# Autodesk Inventor assembly: BoxBeamDBAssembly
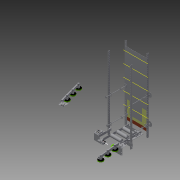
[picture p0: Inventor's stored thumbnail of the model, 180x180]
Saved by Autodesk Inventor 2015 (Build 190159000, 159)
## iProperties
Created: 2015-01-18
Part Number: BoxBeamDBAssembly
Document SubType Name: Assembly
Designer: whitaus15
Author: whitaus15
Title: \\lhssvr02\Homedirs\Robotics Club\CAD Model 2015\Box Beam Drive Base\BoxBeamDBAssembly.stp
Creation Date: 2015-01-17
Sending System: Autodesk Inventor 2015
Preprocessor: ST-DEVELOPER v15.6
## Documents named in this file (21)
- \\lhssvr02\Homedirs\Robotics Club\CAD Model 2015\Box Beam Drive Base\BoxBeamDBAssembly.iam
- \\lhssvr02\Homedirs\Robotics Club\CAD Model 2015\Box Beam Drive Base\Imported Components\BoxBeamDBAssembly\c hannel.ipt
- \\lhssvr02\Homedirs\Robotics Club\CAD Model 2015\Box Beam Drive Base\Imported Components\BoxBeamDBAssembly\Elevator Sprocket with Sprockets.iam
- \\lhssvr02\Homedirs\Robotics Club\CAD Model 2015\Box Beam Drive Base\Imported Components\BoxBeamDBAssembly\c hannel_MIR6.ipt
- \\lhssvr02\Homedirs\Robotics Club\CAD Model 2015\Box Beam Drive Base\Imported Components\BoxBeamDBAssembly\Elevator Sprocket with Sprockets_MIR3.iam
- \\lhssvr02\Homedirs\Robotics Club\CAD Model 2015\Fc Fender Assembly_MIR5.iam
- \\lhssvr02\Homedirs\Robotics Club\CAD Model 2015\Bearing plate version 2.0_MIR4.ipt
- \\lhssvr02\Homedirs\Robotics Club\CAD Model 2015\Fender and Igus.iam
- \\lhssvr02\Homedirs\Robotics Club\CAD Model 2015\Front bar with Motors.iam
- \\lhssvr02\Homedirs\Robotics Club\CAD Model 2015\Fc Fender Assembly_MIR5_MIR.iam
- \\lhssvr02\Homedirs\Robotics Club\CAD Model 2015\Bearing plate version 2.0_MIR4_MIR.ipt
- \\lhssvr02\Homedirs\Robotics Club\CAD Model 2015\Fender and Igus_MIR3.iam
- \\lhssvr02\Homedirs\Robotics Club\CAD Model 2015\Front bar with Motors_MIR.iam
- \\lhssvr02\Homedirs\Robotics Club\CAD Model 2015\Box Beam Drive Base\Conveyor.iam
- \\lhssvr02\Homedirs\Robotics Club\CAD Model 2015\Box Beam Drive Base\Imported Components\BoxBeamDBAssembly\c hannel_MIR.ipt
- \\lhssvr02\Homedirs\Robotics Club\CAD Model 2015\Box Beam Drive Base\Back plate.ipt
- \\lhssvr02\Homedirs\Robotics Club\CAD Model 2015\Box Beam Drive Base\electronics board.iam
- \\lhssvr02\Homedirs\Robotics Club\CAD Model 2015\Elevator parts\Gearbox\Elevator Gearbox Assembly.iam
- \\lhssvr02\Homedirs\Robotics Club\CAD Model 2015\Box Beam Drive Base\Newest\Elevator Shaft Mounts.ipt
- \\lhssvr02\Homedirs\Robotics Club\CAD Model 2015\Elevator parts\Gearbox\S25-60L Aluminum Sprocket (am-0237).0002.ipt
- \\lhssvr02\Homedirs\Robotics Club\CAD Model 2015\Elevator parts\Gearbox\22 tooth sprocket.ipt
## Components (35 placed, 20 different names)
1. c hannel:2 — Angle:2, Mate:12, Mate:19, Mate:22, Mate:23, Mate:53, Mate:57
2. c hannel:3 — Mate:20, Mate:21, Mate:24, Mate:41, Mate:54, Mate:55
3. Elevator Sprocket with Sprockets:1 [sub-assembly] — Mate:30, Mate:61
4. Elevator Sprocket with Sprockets:2 [sub-assembly] — Mate:45, Mate:58, Mate:59
5. c hannel_MIR6:1 — Mate:17, Mate:28, Mate:29, Mate:36, Mate:37, Mate:38
6. Elevator Sprocket with Sprockets_MIR3:1 [sub-assembly] — Mate:25, Mate:64
7. Elevator Sprocket with Sprockets_MIR3:2 [sub-assembly] — Mate:35, Mate:60
8. Fc Fender Assembly_MIR5:1 [sub-assembly] — Flush:10, Flush:11, Mate:15
9. Front bar with Motors:1 [sub-assembly] — Mate:11, Flush:8
10. Fc Fender Assembly_MIR5_MIR:1 [sub-assembly]
11. Bearing plate version 2.0_MIR4_MIR:1 — Mate:8, Mate:9
12. Fender and Igus_MIR3:1 [sub-assembly] — Mate:8, Mate:9
13. Front bar with Motors_MIR:1 [sub-assembly]
14. Back plate:1 — Angle:2, Mate:12, Mate:16, Mate:32, Mate:33, Mate:48, Mate:56
15. Conveyor:1 [sub-assembly] — Mate:11, Flush:8
16. c hannel_MIR:1 — Mate:13, Mate:18, Mate:26, Mate:27, Mate:39
17. electronics board:1 [sub-assembly] — Mate:13, Mate:34, Mate:53, Mate:62, Mate:63
18. Bearing plate version 2.0_MIR4:1
19. Fender and Igus:1 [sub-assembly]
20. Bearing plate version 2.0_MIR4:2 — Flush:10, Flush:11, Mate:15
21. Elevator Gearbox Assembly:1 [sub-assembly] — Mate:16
22. Elevator Shaft Mounts:1 — Mate:18, Mate:26, Mate:27, Mate:30
23. Elevator Shaft Mounts:2 — Mate:17, Mate:28, Mate:29
24. Elevator Shaft Mounts:3 — Mate:19, Mate:22, Mate:23, Mate:25
25. Elevator Shaft Mounts:4 — Mate:20, Mate:21, Mate:24
26. Elevator Shaft Mounts:5 — Mate:32, Mate:33, Mate:34, Mate:35, Mate:39
27. Elevator Shaft Mounts:6 — Mate:36, Mate:37, Mate:38
28. Elevator Shaft Mounts:7 — Mate:41, Mate:54, Mate:55, Mate:58
29. Elevator Shaft Mounts:8 — Mate:45, Mate:48, Mate:56, Mate:57
30. S25-60L Aluminum Sprocket (am-0237).0002:1 — Mate:59
31. S25-60L Aluminum Sprocket (am-0237).0002:2 — Mate:60
32. 22 tooth sprocket:1 — Mate:63
33. 22 tooth sprocket:2 — Mate:62
34. S25-60L Aluminum Sprocket (am-0237).0002:3 — Mate:64
35. S25-60L Aluminum Sprocket (am-0237).0002:4 — Mate:61
## Relationships (48: Mate 44, Flush 3, Angle 1)
- Mate:8: Bearing plate version 2.0_MIR4_MIR:1 ↔ Fender and Igus_MIR3:1
- Mate:9: Bearing plate version 2.0_MIR4_MIR:1 ↔ Fender and Igus_MIR3:1
- Mate:11: Front bar with Motors:1 ↔ Conveyor:1
- Flush:8: Front bar with Motors:1 ↔ Conveyor:1
- Angle:2 (0 deg): c hannel:2 ↔ Back plate:1
- Mate:12: c hannel:2 ↔ Back plate:1
- Mate:13: c hannel_MIR:1 ↔ electronics board:1
- Flush:10: Fc Fender Assembly_MIR5:1 ↔ Bearing plate version 2.0_MIR4:2
- Flush:11: Fc Fender Assembly_MIR5:1 ↔ Bearing plate version 2.0_MIR4:2
- Mate:15: Fc Fender Assembly_MIR5:1 ↔ Bearing plate version 2.0_MIR4:2
- Mate:16: Back plate:1 ↔ Elevator Gearbox Assembly:1
- Mate:17: c hannel_MIR6:1 ↔ Elevator Shaft Mounts:2
- Mate:18: c hannel_MIR:1 ↔ Elevator Shaft Mounts:1
- Mate:19: c hannel:2 ↔ Elevator Shaft Mounts:3
- Mate:20: c hannel:3 ↔ Elevator Shaft Mounts:4
- Mate:21: c hannel:3 ↔ Elevator Shaft Mounts:4
- Mate:22: c hannel:2 ↔ Elevator Shaft Mounts:3
- Mate:23: c hannel:2 ↔ Elevator Shaft Mounts:3
- Mate:24: c hannel:3 ↔ Elevator Shaft Mounts:4
- Mate:25: Elevator Sprocket with Sprockets_MIR3:1 ↔ Elevator Shaft Mounts:3
- Mate:26: c hannel_MIR:1 ↔ Elevator Shaft Mounts:1
- Mate:27: c hannel_MIR:1 ↔ Elevator Shaft Mounts:1
- Mate:28: c hannel_MIR6:1 ↔ Elevator Shaft Mounts:2
- Mate:29: c hannel_MIR6:1 ↔ Elevator Shaft Mounts:2
- Mate:30: Elevator Sprocket with Sprockets:1 ↔ Elevator Shaft Mounts:1
- Mate:32: Back plate:1 ↔ Elevator Shaft Mounts:5
- Mate:33: Back plate:1 ↔ Elevator Shaft Mounts:5
- Mate:34: electronics board:1 ↔ Elevator Shaft Mounts:5
- Mate:35: Elevator Sprocket with Sprockets_MIR3:2 ↔ Elevator Shaft Mounts:5
- Mate:36: c hannel_MIR6:1 ↔ Elevator Shaft Mounts:6
- Mate:37: c hannel_MIR6:1 ↔ Elevator Shaft Mounts:6
- Mate:38: c hannel_MIR6:1 ↔ Elevator Shaft Mounts:6
- Mate:39: c hannel_MIR:1 ↔ Elevator Shaft Mounts:5
- Mate:41: c hannel:3 ↔ Elevator Shaft Mounts:7
- Mate:45: Elevator Sprocket with Sprockets:2 ↔ Elevator Shaft Mounts:8
- Mate:48: Back plate:1 ↔ Elevator Shaft Mounts:8
- Mate:53: c hannel:2 ↔ electronics board:1
- Mate:54: c hannel:3 ↔ Elevator Shaft Mounts:7
- Mate:55: c hannel:3 ↔ Elevator Shaft Mounts:7
- Mate:56: Back plate:1 ↔ Elevator Shaft Mounts:8
- Mate:57: c hannel:2 ↔ Elevator Shaft Mounts:8
- Mate:58: Elevator Sprocket with Sprockets:2 ↔ Elevator Shaft Mounts:7
- Mate:59: Elevator Sprocket with Sprockets:2 ↔ S25-60L Aluminum Sprocket (am-0237).0002:1
- Mate:60: Elevator Sprocket with Sprockets_MIR3:2 ↔ S25-60L Aluminum Sprocket (am-0237).0002:2
- Mate:61: Elevator Sprocket with Sprockets:1 ↔ S25-60L Aluminum Sprocket (am-0237).0002:4
- Mate:62: electronics board:1 ↔ 22 tooth sprocket:2
- Mate:63: electronics board:1 ↔ 22 tooth sprocket:1
- Mate:64: Elevator Sprocket with Sprockets_MIR3:1 ↔ S25-60L Aluminum Sprocket (am-0237).0002:3
